# Autodesk Inventor assembly: Сборка2
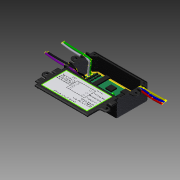
[picture p0: Inventor's stored thumbnail of the model, 180x180]
Saved by Autodesk Inventor 2012 (Build 160160000, 160)
## iProperties
Created: 2009-11-20
Part Number: Сборка2
Document SubType Name: Assembly
Designer: toma
Mass: 20.6369 g
Surface Area: 289.802 cm^2
Volume: 20.6369 cm^3
Density: 1 g/cm^3
Author: toma
## Documents named in this file (7)
- D:\VSS_WORK\VSS_ENERGO\Сумматор light\КД\Сумматор Light\Сборка2.iam
- D:\VSS_WORK\VSS_ENERGO\Сумматор light\КД\Сумматор Light\корпус.ipt
- D:\VSS_WORK\VSS_ENERGO\Сумматор light\КД\Сумматор Light\Сборка платы.iam
- D:\VSS_WORK\VSS_ENERGO\Сумматор light\КД\Сумматор Light\клей.ipt
- D:\VSS_WORK\VSS_ENERGO\Сумматор light\КД\Сумматор Light\контакт.ipt
- D:\Inventor\Сумматор Light\Сборка2\AIP\Провода и кабели\Сборка2.Прокладка кабелей1.iam
- D:\VSS_WORK\VSS_ENERGO\Сумматор light\КД\Сумматор Light\Сборка1.iam
## Components (12 placed, 6 different names)
1. корпус:1 — Совмещение:2, Заподлицо:1, Совмещение:3, Заподлицо:2, Совмещение:4, Совмещение:5, Совмещение:6, Совмещение:8, Совмещение:9, Совмещение:10, Совмещение:11, Совмещение:12, Совмещение:13, Совмещение:14, Совмещение:17, Совмещение:18, Совмещение:19, Совмещение:20, Совмещение:21, Совмещение:22, Совмещение:23, Совмещение:24, Совмещение:25, Совмещение:26, Совмещение:27, Совмещение:28, Совмещение:29, Совмещение:30, Совмещение:31
2. Сборка платы:1 [sub-assembly] — Совмещение:2, Заподлицо:1, Совмещение:3, Заподлицо:3
3. клей:1 — Заподлицо:2, Заподлицо:3, Совмещение:4
4. контакт:1 — Совмещение:5, Совмещение:6, Совмещение:11
5. контакт:2 — Совмещение:8, Совмещение:9, Совмещение:10
6. контакт:3 — Совмещение:12, Совмещение:13, Совмещение:14
7. контакт:4 — Совмещение:18, Совмещение:19, Совмещение:20
8. контакт:5 — Совмещение:17, Совмещение:21, Совмещение:22
9. контакт:6 — Совмещение:23, Совмещение:24, Совмещение:25
10. контакт:7 — Совмещение:26, Совмещение:27, Совмещение:28
11. Прокладка кабелей1 [sub-assembly]
12. Сборка1:1 [sub-assembly] — Совмещение:29, Совмещение:30, Совмещение:31
## Relationships (30: Mate 27, Flush 3)
- Совмещение:2 [Mate]: корпус:1 ↔ Сборка платы:1
- Заподлицо:1 [Flush] (-59.5 mm): корпус:1 ↔ Сборка платы:1
- Совмещение:3 [Mate] (2 mm): корпус:1 ↔ Сборка платы:1
- Заподлицо:2 [Flush] (-34 mm): корпус:1 ↔ клей:1
- Заподлицо:3 [Flush]: Сборка платы:1 ↔ клей:1
- Совмещение:4 [Mate]: корпус:1 ↔ клей:1
- Совмещение:5 [Mate] (25 mm): корпус:1 ↔ контакт:1
- Совмещение:6 [Mate] (0.5 mm): корпус:1 ↔ контакт:1
- Совмещение:8 [Mate] (25 mm): корпус:1 ↔ контакт:2
- Совмещение:9 [Mate] (1.5 mm): корпус:1 ↔ контакт:2
- Совмещение:10 [Mate] (1.8 mm): корпус:1 ↔ контакт:2
- Совмещение:11 [Mate] (-0.5 mm): корпус:1 ↔ контакт:1
- Совмещение:12 [Mate] (25 mm): корпус:1 ↔ контакт:3
- Совмещение:13 [Mate] (1.5 mm): корпус:1 ↔ контакт:3
- Совмещение:14 [Mate] (4.3 mm): корпус:1 ↔ контакт:3
- Совмещение:17 [Mate] (3.2 mm): корпус:1 ↔ контакт:5
- Совмещение:18 [Mate] (1.5 mm): корпус:1 ↔ контакт:4
- Совмещение:19 [Mate] (1.2 mm): корпус:1 ↔ контакт:4
- Совмещение:20 [Mate] (25 mm): корпус:1 ↔ контакт:4
- Совмещение:21 [Mate] (1.5 mm): корпус:1 ↔ контакт:5
- Совмещение:22 [Mate] (25 mm): корпус:1 ↔ контакт:5
- Совмещение:23 [Mate] (24 mm): корпус:1 ↔ контакт:6
- Совмещение:24 [Mate] (1.5 mm): корпус:1 ↔ контакт:6
- Совмещение:25 [Mate] (1.5 mm): корпус:1 ↔ контакт:6
- Совмещение:26 [Mate] (25 mm): корпус:1 ↔ контакт:7
- Совмещение:27 [Mate] (1.5 mm): корпус:1 ↔ контакт:7
- Совмещение:28 [Mate] (3.5 mm): корпус:1 ↔ контакт:7
- Совмещение:29 [Mate]: корпус:1 ↔ Сборка1:1
- Совмещение:30 [Mate] (35 mm): корпус:1 ↔ Сборка1:1
- Совмещение:31 [Mate] (4 mm): корпус:1 ↔ Сборка1:1
